# Autodesk Inventor assembly: botAssemblyVer3
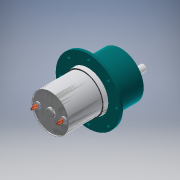
[picture p0: Inventor's stored thumbnail of the model, 180x180]
Saved by Autodesk Inventor 2016 (Build 200138000, 138)
## iProperties
Created: 2016-06-30
Part Number: botAssemblyVer3
Document SubType Name: Assembly
Designer: hesaon
Author: hesaon
## Documents named in this file (5)
- C:\Users\hesaon\Documents\Killer-Bot-2016\AutodeskWorkspace\robot parts revision 3\botAssemblyVer3.iam
- C:\Users\hesaon\Documents\Killer-Bot-2016\AutodeskWorkspace\robot parts revision 3\motor fixture.ipt
- C:\Users\hesaon\Documents\Killer-Bot-2016\AutodeskWorkspace\robotparts revision 2\37D mm metal gearmotor.ipt
- C:\Users\hesaon\Documents\Killer-Bot-2016\AutodeskWorkspace\machine screws and nuts\machineScrew3x10.ipt
- C:\Users\hesaon\Documents\Killer-Bot-2016\AutodeskWorkspace\machine screws and nuts\washer3mm.ipt
## Components (14 placed, 4 different names)
1. motor fixture:1 — Insert:1, Insert:2, Insert:3, Insert:4, Insert:5, Insert:6, Insert:7, Insert:8
2. 37D mm metal gearmotor:1 — Insert:1, Insert:2
3. machineScrew3x10:1 — Insert:9
4. machineScrew3x10:2 — Insert:10
5. machineScrew3x10:3 — Insert:11
6. machineScrew3x10:4 — Insert:12
7. machineScrew3x10:5 — Insert:13
8. machineScrew3x10:6 — Insert:14
9. washer3mm:1 — Insert:3, Insert:11
10. washer3mm:2 — Insert:4, Insert:10
11. washer3mm:3 — Insert:5, Insert:9
12. washer3mm:4 — Insert:6, Insert:12
13. washer3mm:5 — Insert:7, Insert:13
14. washer3mm:6 — Insert:8, Insert:14
## Relationships (14: Insert 14)
- Insert:1: motor fixture:1 ↔ 37D mm metal gearmotor:1
- Insert:2: motor fixture:1 ↔ 37D mm metal gearmotor:1
- Insert:3: motor fixture:1 ↔ washer3mm:1
- Insert:4: motor fixture:1 ↔ washer3mm:2
- Insert:5: motor fixture:1 ↔ washer3mm:3
- Insert:6: motor fixture:1 ↔ washer3mm:4
- Insert:7: motor fixture:1 ↔ washer3mm:5
- Insert:8: motor fixture:1 ↔ washer3mm:6
- Insert:9: machineScrew3x10:1 ↔ washer3mm:3
- Insert:10: machineScrew3x10:2 ↔ washer3mm:2
- Insert:11: machineScrew3x10:3 ↔ washer3mm:1
- Insert:12: machineScrew3x10:4 ↔ washer3mm:4
- Insert:13: machineScrew3x10:5 ↔ washer3mm:5
- Insert:14: machineScrew3x10:6 ↔ washer3mm:6
